# Autodesk Inventor assembly: assem_linact_thumb_rod
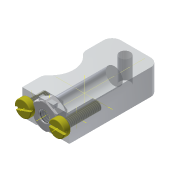
[picture p0: Inventor's stored thumbnail of the model, 180x180]
Saved by Autodesk Inventor 2014 (Build 180170000, 170)
## iProperties
Created: 2015-06-01
Part Number: assem_linact_thumb_rod
Document SubType Name: Assembly
Designer: Martin
Author: Martin
## Documents named in this file (5)
- C:\Users\Martin\Dropbox\biohand-mec\biohand_v1\fingers\thumb\assem_linact_thumb_rod.iam
- C:\Users\Martin\Dropbox\biohand-mec\biohand_v1\fingers\thumb\linact_thumb_rod.ipt
- C:\Users\Martin\Dropbox\biohand-mec\biohand_v1\misc\m3_nut.ipt
- C:\Users\Martin\Dropbox\biohand-mec\biohand_v1\misc\m2_8_screw.ipt
- C:\Users\Martin\Dropbox\biohand-mec\biohand_v1\misc\m2_4_screw.ipt
## Components (4 placed, 4 different names)
1. linact_thumb_rod:1 — Insert:1, Mate:1, Insert:3, Insert:4, Insert:5
2. m3_nut:1 — Insert:1, Mate:1
3. m2_8_screw:1 — Insert:3
4. m2_4_screw:1 — Insert:4, Insert:5
## Relationships (5: Insert 4, Mate 1)
- Insert:1: linact_thumb_rod:1 ↔ m3_nut:1
- Mate:1: linact_thumb_rod:1 ↔ m3_nut:1
- Insert:3: linact_thumb_rod:1 ↔ m2_8_screw:1
- Insert:4: linact_thumb_rod:1 ↔ m2_4_screw:1
- Insert:5: linact_thumb_rod:1 ↔ m2_4_screw:1
